# Autodesk Inventor assembly: Arm 2.0 Assembly
(part 2 of 2)
- Mate:876: AA037:1 ↔ ISO 4018 M5 x 25:36
- Flush:25 (-9 mm): AA037:1 ↔ ISO 4018 M5 x 25:39
- Flush:26 (9 mm): AA037:1 ↔ ISO 4018 M5 x 25:38
- Mate:877: AA016b:1 ↔ ISO 4018 M5 x 25:37
- Mate:878: AA016b:1 ↔ ISO 4018 M5 x 25:36
- Mate:879: AA034:1 ↔ ISO 4018 M5 x 25:42
- Mate:880: AA034:1 ↔ ISO 4018 M5 x 25:41
- Mate:881: AA034:1 ↔ ISO 4018 M5 x 25:43
- Mate:882: AA034:1 ↔ ISO 4018 M5 x 25:40
- Mate:883: AA034:1 ↔ ISO 4018 M5 x 25:40
- Mate:884: AA034:1 ↔ ISO 4018 M5 x 25:43
- Mate:885: AA034:1 ↔ ISO 4018 M5 x 25:42
- Mate:886: AA034:1 ↔ ISO 4018 M5 x 25:41
- Mate:887: 4mm mounting hub:1 ↔ AASG01
- Mate:888: AASG01 ↔ ISO 7045 H M3 x 12 - 4.8 - H:9
- Mate:889: AASG01 ↔ ISO 7045 H M3 x 12 - 4.8 - H:8
- Mate:890: AASG01 ↔ ISO 7045 H M3 x 12 - 4.8 - H:8
- Mate:891: AASG01 ↔ ISO 7045 H M3 x 12 - 4.8 - H:9
- Mate:892: AA044:2 ↔ ISO 7045 H M3 x 8 - 4.8 - H:12
- Mate:893: AA044:2 ↔ ISO 7045 H M3 x 8 - 4.8 - H:12
- Mate:894: uxcell 12V 5RPM 8mm Worm Gear Motor:1 ↔ 8mm Hub:10
- Mate:895: AA001c:1 ↔ 8mm Hub:10
- Mate:896: 8mm Hub:10 ↔ AASG02
- Mate:897: AASG02 ↔ ISO 7045 H M3 x 8 - 4.8 - H:13
- Mate:898: AASG02 ↔ ISO 7045 H M3 x 8 - 4.8 - H:14
- Mate:899: AASG02 ↔ ISO 7045 H M3 x 8 - 4.8 - H:15
- Mate:900: AASG02 ↔ ISO 7045 H M3 x 8 - 4.8 - H:13
- Mate:901: AASG02 ↔ ISO 7045 H M3 x 8 - 4.8 - H:14
- Mate:902: AASG02 ↔ ISO 7045 H M3 x 8 - 4.8 - H:15
- Mate:903: uxcell 12V 5RPM 8mm Worm Gear Motor:1 ↔ ISO 4762 M4 x 10:1
- Mate:904: uxcell 12V 5RPM 8mm Worm Gear Motor:1 ↔ ISO 4762 M4 x 10:2
- Mate:905: AA001c:1 ↔ ISO 4762 M4 x 10:1
- Mate:906: AA001c:1 ↔ ISO 4762 M4 x 10:2
- Mate:907: 12V DC Motor 378-1:6 ↔ ISO 7045 H M3 x 8 - 4.8 - H:17
- Mate:908: 12V DC Motor 378-1:6 ↔ ISO 7045 H M3 x 8 - 4.8 - H:16
- Mate:909: AA005b:1 ↔ ISO 7045 H M3 x 8 - 4.8 - H:17
- Mate:910: AA005b:1 ↔ ISO 7045 H M3 x 8 - 4.8 - H:16
- Mate:911: 8mm Hub:6 ↔ ISO 7045 H M3 x 12 - 4.8 - H:10
- Mate:912: 8mm Hub:6 ↔ ISO 7045 H M3 x 12 - 4.8 - H:12
- Mate:913: 8mm Hub:6 ↔ ISO 7045 H M3 x 12 - 4.8 - H:11
- Mate:914: 8mm Hub:6 ↔ ISO 7045 H M3 x 12 - 4.8 - H:10
- Mate:915: 8mm Hub:6 ↔ ISO 7045 H M3 x 12 - 4.8 - H:11
- Mate:916: 8mm Hub:6 ↔ ISO 7045 H M3 x 12 - 4.8 - H:12
- Mate:917: AASG04 ↔ ISO 7045 H M3 x 12 - 4.8 - H:14
- Mate:918: AASG04 ↔ ISO 7045 H M3 x 12 - 4.8 - H:15
- Mate:919: AASG04 ↔ ISO 7045 H M3 x 12 - 4.8 - H:13
- Mate:920: AASG04 ↔ ISO 7045 H M3 x 12 - 4.8 - H:13
- Mate:921: AASG04 ↔ ISO 7045 H M3 x 12 - 4.8 - H:14
- Mate:922: AASG04 ↔ ISO 7045 H M3 x 12 - 4.8 - H:15
- Mate:923: 12V DC Motor 378-1:7 ↔ ISO 7045 H M3 x 8 - 4.8 - H:18
- Mate:924: 12V DC Motor 378-1:7 ↔ ISO 7045 H M3 x 8 - 4.8 - H:19
- Mate:925: AA008d:1 ↔ ISO 7045 H M3 x 8 - 4.8 - H:18
- Mate:926: AA008d:1 ↔ ISO 7045 H M3 x 8 - 4.8 - H:19
- Mate:927: AA010b:1 ↔ ISO 7045 H M3 x 12 - 4.8 - H:21
- Mate:928: AA010b:1 ↔ ISO 7045 H M3 x 12 - 4.8 - H:20
- Mate:929: AA010b:1 ↔ ISO 7045 H M3 x 12 - 4.8 - H:16
- Mate:930: AA010b:1 ↔ ISO 7045 H M3 x 12 - 4.8 - H:19
- Mate:931: AA010b:1 ↔ ISO 7045 H M3 x 12 - 4.8 - H:18
- Mate:932: AA010b:1 ↔ ISO 7045 H M3 x 12 - 4.8 - H:17
- Mate:933: 8mm Hub:3 ↔ ISO 7045 H M3 x 12 - 4.8 - H:19
- Mate:934: 8mm Hub:3 ↔ ISO 7045 H M3 x 12 - 4.8 - H:17
- Mate:935: 8mm Hub:3 ↔ ISO 7045 H M3 x 12 - 4.8 - H:18
- Mate:936: 8mm Hub:3 ↔ ISO 7045 H M3 x 12 - 4.8 - H:16
- Mate:937: 8mm Hub:3 ↔ ISO 7045 H M3 x 12 - 4.8 - H:20
- Mate:938: 8mm Hub:3 ↔ ISO 7045 H M3 x 12 - 4.8 - H:21
- Mate:939: AA036:1 ↔ ISO 4018 M5 x 25:33
- Mate:940: AASG03 ↔ ISO 7045 H M3 x 12 - 4.8 - H:24
- Mate:941: AASG03 ↔ ISO 7045 H M3 x 12 - 4.8 - H:23
- Mate:942: AASG03 ↔ ISO 7045 H M3 x 12 - 4.8 - H:22
- Mate:943: AASG03 ↔ ISO 7045 H M3 x 12 - 4.8 - H:22
- Mate:944: AASG03 ↔ ISO 7045 H M3 x 12 - 4.8 - H:23
- Mate:945: AASG03 ↔ ISO 7045 H M3 x 12 - 4.8 - H:24
- Mate:946: uxcell 12V 6RPM 6mm Worm Gear Motor:1 ↔ ISO 4762 M4 x 10:3
- Mate:947: uxcell 12V 6RPM 6mm Worm Gear Motor:1 ↔ ISO 4762 M4 x 10:4
- Mate:948: AA010b:1 ↔ ISO 4762 M4 x 10:4
- Mate:949: AA010b:1 ↔ ISO 4762 M4 x 10:3
- Mate:950: AA037:1 ↔ ISO 7045 H M3 x 8 - 4.8 - H:21
- Mate:951: AA037:1 ↔ ISO 7045 H M3 x 8 - 4.8 - H:20
- Mate:952: AA037:1 ↔ ISO 7045 H M3 x 8 - 4.8 - H:21
- Mate:953: AA037:1 ↔ ISO 7045 H M3 x 8 - 4.8 - H:20
- Mate:958: AASG07 ↔ ISO 7045 H M3 x 8 - 4.8 - H:25
- Mate:959: AASG07 ↔ ISO 7045 H M3 x 8 - 4.8 - H:26
- Mate:960: AASG07 ↔ ISO 7045 H M3 x 8 - 4.8 - H:24
- Mate:961: AASG07 ↔ ISO 7045 H M3 x 8 - 4.8 - H:26
- Mate:962: AASG07 ↔ ISO 7045 H M3 x 8 - 4.8 - H:25
- Mate:963: AASG07 ↔ ISO 7045 H M3 x 8 - 4.8 - H:24
- Mate:964: AA034:1 ↔ ISO 7045 H M3 x 8 - 4.8 - H:28
- Mate:965: AA034:1 ↔ ISO 7045 H M3 x 8 - 4.8 - H:27
- Mate:966: AA034:1 ↔ ISO 7045 H M3 x 8 - 4.8 - H:29
- Mate:967: AA034:1 ↔ ISO 7045 H M3 x 8 - 4.8 - H:30
- Mate:968: AA034:1 ↔ ISO 7045 H M3 x 8 - 4.8 - H:32
- Mate:969: AA034:1 ↔ ISO 7045 H M3 x 8 - 4.8 - H:31
- Mate:970: AA034:1 ↔ ISO 7045 H M3 x 8 - 4.8 - H:30
- Mate:971: AA034:1 ↔ ISO 7045 H M3 x 8 - 4.8 - H:29
- Mate:972: AA034:1 ↔ ISO 7045 H M3 x 8 - 4.8 - H:27
- Mate:973: AA034:1 ↔ ISO 7045 H M3 x 8 - 4.8 - H:28
- Mate:974: AA034:1 ↔ ISO 7045 H M3 x 8 - 4.8 - H:32
- Mate:975: AA034:1 ↔ ISO 7045 H M3 x 8 - 4.8 - H:31
- Mate:976: AA014:2 ↔ ISO 4017 M5 x 20:6
- Mate:977: AA014:2 ↔ ISO 4017 M5 x 20:5
- Mate:978: AA014:2 ↔ ISO 4017 M5 x 20:4
- Mate:979: AA014:2 ↔ ISO 4017 M5 x 20:5
- Mate:980: AA014:2 ↔ ISO 4017 M5 x 20:4
- Mate:981: AA014:2 ↔ ISO 4017 M5 x 20:6
- Mate:982: AA045:2 ↔ ISO 4035 M5:6
- Mate:983: AA045:2 ↔ ISO 4035 M5:5
- Mate:984: ISO 4035 M5:6 ↔ ISO 4018 M5 x 25:40
- Mate:985: ISO 4035 M5:5 ↔ ISO 4018 M5 x 25:42
- Mate:986: AA045:2 ↔ ISO 4035 M5:7
- Mate:987: AA045:2 ↔ ISO 4035 M5:8
- Mate:988: ISO 4035 M5:8 ↔ ISO 4018 M5 x 25:41
- Mate:989: ISO 4035 M5:7 ↔ ISO 4018 M5 x 25:43
- Mate:990: 8mm Hub:11 ↔ CNS 4320 M8 x 100:1
- Mate:991: 8mm Hub:11 ↔ CNS 4320 M8 x 100:1
- Mate:992: AA050:1 ↔ CNS 4320 M8 x 100:1
- Mate:994: AA050:1 ↔ 4mm mounting hub:3
- Mate:995: AA050:1 ↔ 8mm Hub:11
- Mate:997: 4mm mounting hub:3 ↔ ISO 7045 H M3 x 8 - 4.8 - H:22
- Mate:999: AA050:1 ↔ 8mm Hub:11
- Mate:1000: 4mm mounting hub:3 ↔ ISO 7045 H M3 x 8 - 4.8 - H:23
- Mate:1001: AA050:1 ↔ 4mm mounting hub:3
- Mate:1002: AA050:1 ↔ ISO 7045 H M3 x 12 - 4.8 - H:25
- Mate:1003: AA050:1 ↔ ISO 7045 H M3 x 12 - 4.8 - H:26
- Mate:1004: AA050:1 ↔ ISO 7045 H M3 x 12 - 4.8 - H:27
- Mate:1005: 8mm Hub:11 ↔ ISO 7045 H M3 x 12 - 4.8 - H:26
- Mate:1006: 8mm Hub:11 ↔ ISO 7045 H M3 x 12 - 4.8 - H:27
- Mate:1007 (3 mm): 22x8x8mm Bearing:8 ↔ 8mm Hub:11
- Mate:1008: 8mm Hub:12 ↔ AS 1110 - Metric M8 x 150:2
- Mate:1009: 8mm Hub:12 ↔ AS 1110 - Metric M8 x 150:2
- Mate:1011: 8mm Hub:12 ↔ AASG06
- Mate:1012: 8mm Hub:12 ↔ AASG06
- Mate:1013: AASG06 ↔ ISO 7045 H M3 x 8 - 4.8 - H:33
- Mate:1014: AASG06 ↔ ISO 7045 H M3 x 8 - 4.8 - H:34
- Mate:1015: AASG06 ↔ ISO 7045 H M3 x 8 - 4.8 - H:34
- Mate:1016: 4mm mounting hub:7 ↔ AASG06
- Mate:1017: AASG06 ↔ ISO 7045 H M3 x 8 - 4.8 - H:33
- Mate:1018: 8mm Hub:12 ↔ ISO 7045 H M3 x 12 - 4.8 - H:29
- Mate:1019: 8mm Hub:12 ↔ ISO 7045 H M3 x 12 - 4.8 - H:28
- Mate:1020: 8mm Hub:12 ↔ ISO 7045 H M3 x 12 - 4.8 - H:30
- Mate:1021: 8mm Hub:12 ↔ ISO 7045 H M3 x 12 - 4.8 - H:28
- Mate:1022: 8mm Hub:12 ↔ ISO 7045 H M3 x 12 - 4.8 - H:29
- Mate:1023: 8mm Hub:12 ↔ ISO 7045 H M3 x 12 - 4.8 - H:30
- Mate:1024: AA035:1 ↔ ISO 4018 M5 x 40:4
- Mate:1025: AA035:1 ↔ ISO 4018 M5 x 40:3
- Flush:27: ISO 4018 M5 x 40:1 ↔ ISO 4018 M5 x 40:4
- Flush:28: ISO 4018 M5 x 40:3 ↔ ISO 4018 M5 x 40:4
- Mate:1026: ISO 4035 M5:9 ↔ ISO 4018 M5 x 40:4
- Mate:1027: ISO 4035 M5:10 ↔ ISO 4018 M5 x 40:3
- Mate:1028: AA035:1 ↔ ISO 4035 M5:9
- Mate:1029: AA035:1 ↔ ISO 4035 M5:10
- Mate:1030: AA008c:1 ↔ AA008d:1
- Mate:1031: AA008c:1 ↔ ISO 4018 M5 x 40:4
- Mate:1032: AA008c:1 ↔ ISO 4018 M5 x 40:3
- Mate:1033: AA008c:1 ↔ AA008d:1
